# Autodesk Inventor assembly: Housing_Assembly_V4
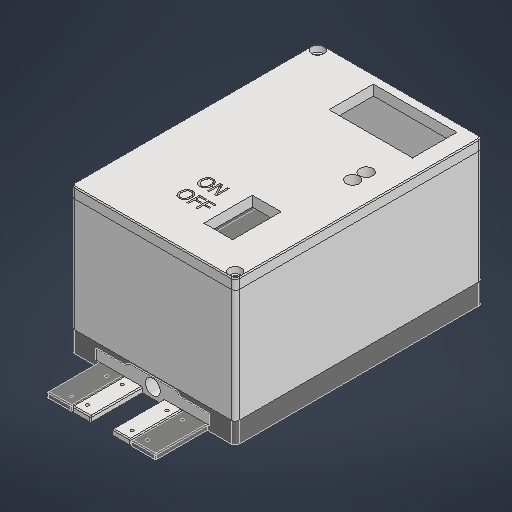
[picture p0: Inventor's stored thumbnail of the model, 512x512]
Saved by Autodesk Inventor 2026.2 (Build 302298000, 298)
## iProperties
Created: 2026-03-15
Part Number: Housing_Assembly_V4
Document SubType Name: Assembly
Designer: vckot
Author: vckot
## Documents named in this file (17)
- C:\Users\vckot\OneDrive\Documents\Vaibhav\capstone\CAD_files\Housing_Assembly_V4.iam
- C:\Users\vckot\OneDrive\Documents\Vaibhav\capstone\CAD_files\PCB_Housing\PCB_Housing_01_V4.ipt
- C:\Users\vckot\OneDrive\Documents\Vaibhav\capstone\CAD_files\Batteries\Battery_Small.ipt
- C:\Users\vckot\OneDrive\Documents\Vaibhav\capstone\CAD_files\Motor\Adafruit_1528_4699_ND.ipt
- C:\Users\vckot\OneDrive\Documents\Vaibhav\capstone\CAD_files\Motor_Valve\Adafruit_1528-4663-ND.ipt
- C:\Users\vckot\OneDrive\Documents\Vaibhav\capstone\CAD_files\Pipe_Connectors\Adafruit_4662.ipt
- C:\Users\vckot\OneDrive\Documents\Vaibhav\capstone\CAD_files\Snap_Switch\Snap_Switch_Assembly.iam
- C:\Users\vckot\OneDrive\Documents\Vaibhav\capstone\CAD_files\PCB_Housing\PCB_Housing_02_V4.ipt
- C:\Users\vckot\OneDrive\Documents\Vaibhav\capstone\CAD_files\PCB_Housing\PCB_Housing_03_V4.ipt
- C:\Users\vckot\OneDrive\Documents\Vaibhav\capstone\CAD_files\PCB_Housing\PCB_Housing_04_V4.ipt
- C:\Users\vckot\OneDrive\Documents\Vaibhav\capstone\CAD_files\PCB_Housing\TourniquetPCBV1_Updated\TourniquetPCBV1_Updated\TourniquetPCBV1_Updated.iam
- C:\Users\vckot\OneDrive\Documents\Vaibhav\capstone\CAD_files\PCB_Housing\PCB_Housing_05_V4.ipt
- C:\Users\vckot\OneDrive\Documents\Vaibhav\capstone\CAD_files\7_Segment_Display\7_Seg_Display_TM1637.ipt
- C:\Users\vckot\Downloads\91290A120_Black-Oxide Alloy Steel Socket Head Screw\91290A120_Black-Oxide Alloy Steel Socket Head Screw\91290A120_Black-Oxide Alloy Steel Socket Head Screw.ipt
- C:\Users\vckot\OneDrive\Documents\Vaibhav\capstone\CAD_files\PCB_Housing\PCB_Housing_07_V4.ipt
- C:\Users\vckot\OneDrive\Documents\Vaibhav\capstone\CAD_files\PCB_Housing\PCB_Housing_06_V4.ipt
- C:\Users\vckot\OneDrive\Documents\Vaibhav\capstone\CAD_files\Tourniquet_Rails\Tourniquet_Rail_01_V4.ipt
## Components (17 placed, 16 different names)
1. PCB_Housing_01_V4:1 — Flush:1, Flush:2, Flush:3, Mate:1, Flush:4, Flush:5, Mate:2, Angle:1, Mate:11, Mate:13, Mate:14, Flush:7, Flush:8, Mate:17, Mate:25, Flush:14, Mate:26, Flush:15, Flush:16
2. Battery_Small:1 — Mate:1, Flush:4, Flush:5, Flush:6, Mate:3, Mate:15
3. Adafruit_1528_4699_ND:1 — Mate:2, Flush:6, Mate:3, Mate:4, Mate:5
4. Adafruit_1528-4663-ND:1 — Mate:4, Mate:5, Angle:1, Mate:6, Mate:7, Angle:2
5. Adafruit_4662:1 — Mate:6, Mate:7, Angle:2
6. Adafruit_4662:2 — Mate:12, Mate:13
7. Snap_Switch_Assembly:1 [sub-assembly] — Mate:9, Mate:10, Mate:11, Mate:12
8. PCB_Housing_02_V4:1 — Mate:14, Mate:15, Mate:16, Mate:18, Flush:9, Flush:10, Mate:19, Flush:11, Mate:20
9. PCB_Housing_03_V4:1 — Flush:7, Flush:8, Mate:17, Mate:9, Mate:10, Mate:16, Angle:3, Angle:4, Flush:12, Flush:13, Mate:24
10. PCB_Housing_04_V4:1 — Mate:18, Flush:9, Flush:10, Mate:21
11. TourniquetPCBV1_Updated:1 [sub-assembly] — Angle:3, Angle:4, Angle:5, Mate:21
12. PCB_Housing_05_V4:1 — Mate:19, Flush:11, Mate:20
13. 7_Seg_Display_TM1637:1 — Angle:5
14. 91290A120_Black-Oxide Alloy Steel Socket Head Screw:2
15. PCB_Housing_06_V4:1 — Flush:12, Flush:13, Mate:24
16. PCB_Housing_07_V4:1 — Mate:25, Flush:14, Mate:26, Mate:27
17. Tourniquet_Rail_01_V4:1 — Flush:15, Flush:16, Mate:27
## Relationships (47: Mate 26, Flush 16, Angle 5)
- Flush:1: PCB_Housing_01_V4:1
- Flush:2: PCB_Housing_01_V4:1
- Flush:3: PCB_Housing_01_V4:1
- Mate:1: PCB_Housing_01_V4:1 ↔ Battery_Small:1
- Flush:4 (2.5 mm): PCB_Housing_01_V4:1 ↔ Battery_Small:1
- Flush:5 (2.5 mm): PCB_Housing_01_V4:1 ↔ Battery_Small:1
- Mate:2 (1 mm): PCB_Housing_01_V4:1 ↔ Adafruit_1528_4699_ND:1
- Flush:6 (2 mm): Battery_Small:1 ↔ Adafruit_1528_4699_ND:1
- Mate:3 (18 mm): Battery_Small:1 ↔ Adafruit_1528_4699_ND:1
- Mate:4: Adafruit_1528_4699_ND:1 ↔ Adafruit_1528-4663-ND:1
- Mate:5 (1 mm): Adafruit_1528_4699_ND:1 ↔ Adafruit_1528-4663-ND:1
- Angle:1 (180 deg): PCB_Housing_01_V4:1 ↔ Adafruit_1528-4663-ND:1
- Mate:6: Adafruit_1528-4663-ND:1 ↔ Adafruit_4662:1
- Mate:7 (5 mm): Adafruit_1528-4663-ND:1 ↔ Adafruit_4662:1
- Angle:2 (45 deg): Adafruit_1528-4663-ND:1 ↔ Adafruit_4662:1
- Mate:9: Snap_Switch_Assembly:1 ↔ PCB_Housing_03_V4:1
- Mate:10: Snap_Switch_Assembly:1 ↔ PCB_Housing_03_V4:1
- Mate:11: PCB_Housing_01_V4:1 ↔ Snap_Switch_Assembly:1
- Mate:12: Adafruit_4662:2 ↔ Snap_Switch_Assembly:1
- Mate:13: PCB_Housing_01_V4:1 ↔ Adafruit_4662:2
- Mate:14: PCB_Housing_01_V4:1 ↔ PCB_Housing_02_V4:1
- Mate:15: Battery_Small:1 ↔ PCB_Housing_02_V4:1
- Mate:16: PCB_Housing_02_V4:1 ↔ PCB_Housing_03_V4:1
- Flush:7: PCB_Housing_01_V4:1 ↔ PCB_Housing_03_V4:1
- Flush:8: PCB_Housing_01_V4:1 ↔ PCB_Housing_03_V4:1
- Mate:17: PCB_Housing_01_V4:1 ↔ PCB_Housing_03_V4:1
- Mate:18: PCB_Housing_02_V4:1 ↔ PCB_Housing_04_V4:1
- Flush:9: PCB_Housing_02_V4:1 ↔ PCB_Housing_04_V4:1
- Flush:10: PCB_Housing_02_V4:1 ↔ PCB_Housing_04_V4:1
- Angle:3 (0 deg): PCB_Housing_03_V4:1 ↔ TourniquetPCBV1_Updated:1
- Angle:4 (0 deg): PCB_Housing_03_V4:1 ↔ TourniquetPCBV1_Updated:1
- Mate:19: PCB_Housing_02_V4:1 ↔ PCB_Housing_05_V4:1
- Flush:11: PCB_Housing_02_V4:1 ↔ PCB_Housing_05_V4:1
- Mate:20 (2.5 mm): PCB_Housing_02_V4:1 ↔ PCB_Housing_05_V4:1
- Angle:5 (0 deg): TourniquetPCBV1_Updated:1 ↔ 7_Seg_Display_TM1637:1
- Mate:21: PCB_Housing_04_V4:1 ↔ TourniquetPCBV1_Updated:1
- [Mate]: PCB_Housing_01_V4:1 ↔ 91290A120_Black-Oxide Alloy Steel Socket Head Screw:2
- [Mate]: PCB_Housing_01_V4:1 ↔ 91290A120_Black-Oxide Alloy Steel Socket Head Screw:2
- Flush:12: PCB_Housing_03_V4:1 ↔ PCB_Housing_06_V4:1
- Flush:13: PCB_Housing_03_V4:1 ↔ PCB_Housing_06_V4:1
- Mate:24: PCB_Housing_03_V4:1 ↔ PCB_Housing_06_V4:1
- Mate:25: PCB_Housing_01_V4:1 ↔ PCB_Housing_07_V4:1
- Flush:14: PCB_Housing_01_V4:1 ↔ PCB_Housing_07_V4:1
- Mate:26: PCB_Housing_01_V4:1 ↔ PCB_Housing_07_V4:1
- Flush:15: PCB_Housing_01_V4:1 ↔ Tourniquet_Rail_01_V4:1
- Flush:16: PCB_Housing_01_V4:1 ↔ Tourniquet_Rail_01_V4:1
- Mate:27: PCB_Housing_07_V4:1 ↔ Tourniquet_Rail_01_V4:1
